# Autodesk Inventor assembly: ASY PNS-0210 frame right floor
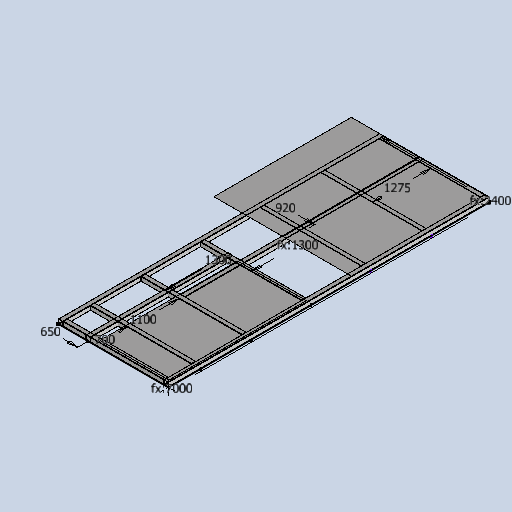
[picture p0: Inventor's stored thumbnail of the model, 512x512]
Saved by Autodesk Inventor 2025 (Build 290162010, 162A)
## iProperties
Created: 2025-03-15
Part Number: ASY PNS-0210 frame right floor
Document SubType Name: Assembly
Designer: admin
_SolveAssemblyDoc: Frame Generator Solve Assembly
_Version: 25.0.0
Author: admin
## Documents named in this file (4)
- C:\Users\admin\YandexDisk-badmisterfox\home pc\Inventor\PNS-Panaevsk\ASY PNS-0210 frame right floor.iam
- C:\Users\admin\YandexDisk-badmisterfox\home pc\Inventor\PNS-Panaevsk\PNS-0210 frame right floor Sketch.ipt
- C:\Users\admin\YandexDisk-badmisterfox\home pc\Inventor\PNS-Panaevsk\ASY PNS-0210 frame right floor\Frame\Frame 1742033625963.iam
- C:\Users\admin\YandexDisk-badmisterfox\home pc\Inventor\PNS-Panaevsk\PNS-0111 floor sheet 2.ipt
## Components (5 placed, 3 different names)
1. PNS-0210 frame right floor Sketch:1
2. PNS-0111 floor sheet 2:2
3. PNS-0111 floor sheet 2:3
4. PNS-0111 floor sheet 2:1
5. Frame 1742033625963:1 [sub-assembly]
## Relationships (2: Mate 2)
- [Mate]: PNS-0111 floor sheet 2:2 ↔ Frame 1742033625963:1
- [Mate]: PNS-0111 floor sheet 2:3 ↔ Frame 1742033625963:1
